# Autodesk Inventor assembly: bat_mount_v3
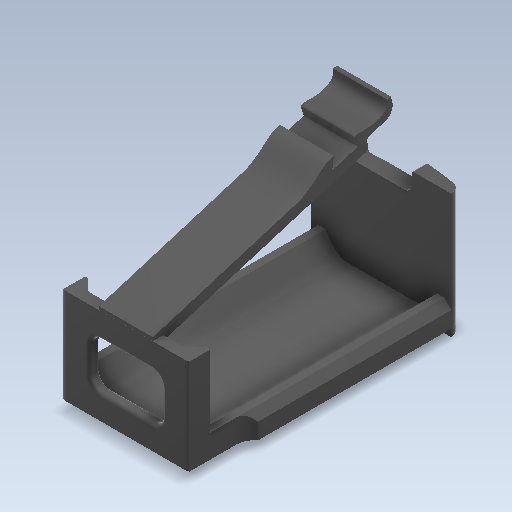
[picture p0: Inventor's stored thumbnail of the model, 512x512]
Saved by Autodesk Inventor 2020 (Build 240168000, 168)
## iProperties
Created: 2024-02-13
Part Number: bat_mount_v3
Document SubType Name: Assembly
Designer: 4s
Author: 4s
## Documents named in this file (3)
- C:\Users\4s\Documents\Inventor models\Asterisk\robot_v2\Bat_mount\bat_mount_v3.iam
- C:\Users\4s\Documents\Inventor models\Asterisk\robot_v2\Bat_mount\bat_mount003.ipt
- C:\Users\4s\Documents\Inventor models\Asterisk\robot_v2\Bat_mount\bat_lock03.ipt
## Components (2 placed, 2 different names)
1. bat_mount003:1 — Заподлицо:1, Совмещение:1, Заподлицо:2, Совмещение:2, Заподлицо:4, Заподлицо:5, Совмещение:5
2. bat_lock03:1 — Заподлицо:4, Заподлицо:5, Совмещение:5
## Relationships (7: Flush 4, Mate 3)
- Заподлицо:1 [Flush]: bat_mount003:1
- Совмещение:1 [Mate]: bat_mount003:1
- Заподлицо:2 [Flush]: bat_mount003:1
- Совмещение:2 [Mate]: bat_mount003:1
- Заподлицо:4 [Flush] (10 mm): bat_mount003:1 ↔ bat_lock03:1
- Заподлицо:5 [Flush] (0.05 mm): bat_mount003:1 ↔ bat_lock03:1
- Совмещение:5 [Mate] (-5 mm): bat_mount003:1 ↔ bat_lock03:1
